# Autodesk Inventor assembly: Front_Panel_BASE_STATION_Assembly
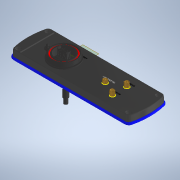
[picture p0: Inventor's stored thumbnail of the model, 180x180]
Saved by Autodesk Inventor 2022 (Build 260153000, 153)
## iProperties
Created: 2021-04-26
Part Number: Front_Panel_BASE_STATION_Assembly
Document SubType Name: Assembly
Designer: lgnds
Author: lgnds
## Documents named in this file (5)
- C:\Users\Viktor\Documents\GitHub\MARV-Hardware-Mechanical\GPS Base Station\Front_Panel\Front_Panel_BASE_STATION_Assembly.iam
- C:\Users\Viktor\Documents\GitHub\MARV-Hardware-Mechanical\GPS Base Station\Front_Panel\Panel\1009799_3D_Front_WaveRunner.ipt
- C:\Users\Viktor\Documents\GitHub\MARV-Hardware-Mechanical\GPS Base Station\Back_Panel\Connectors\LAIRD_080-0014.ipt
- C:\Users\Viktor\Documents\GitHub\MARV-Hardware-Mechanical\GPS Base Station\Back_Panel\Panel\DI 1600.ipt
- C:\Users\Viktor\Documents\GitHub\MARV-Hardware-Mechanical\GPS Base Station\Front_Panel\Connectors\PX0844A0M50A\px0844-a-0m50-b.iam
## Components (6 placed, 4 different names)
1. 1009799_3D_Front_WaveRunner:1 — Rigid:1, Rigid:2, Rigid:3, Rigid:4, Rigid:5
2. LAIRD_080-0014:1 — Rigid:2
3. LAIRD_080-0014:2 — Rigid:3
4. LAIRD_080-0014:3 — Rigid:4
5. DI 1600:1 — Rigid:1
6. px0844-a-0m50-b:1 [sub-assembly] — Rigid:5
## Relationships (5: WeldJoint 5)
- Rigid:1 [WeldJoint]: 1009799_3D_Front_WaveRunner:1 ↔ DI 1600:1
- Rigid:2 [WeldJoint]: 1009799_3D_Front_WaveRunner:1 ↔ LAIRD_080-0014:1
- Rigid:3 [WeldJoint]: 1009799_3D_Front_WaveRunner:1 ↔ LAIRD_080-0014:2
- Rigid:4 [WeldJoint]: 1009799_3D_Front_WaveRunner:1 ↔ LAIRD_080-0014:3
- Rigid:5 [WeldJoint]: 1009799_3D_Front_WaveRunner:1 ↔ px0844-a-0m50-b:1
